# Autodesk Inventor assembly: Assembly
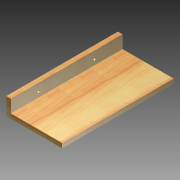
[picture p0: Inventor's stored thumbnail of the model, 180x180]
Saved by Autodesk Inventor 2012 (Build 160160000, 160)
## iProperties
Created: 2013-12-06
Part Number: Assembly
Document SubType Name: Assembly
Designer: PADIAUMESH
Author: PADIAUMESH
## Documents named in this file (3)
- C:\Users\PADIAUMESH\git\AbilityOne\CAD\Assembly.iam
- C:\Users\PADIAUMESH\git\AbilityOne\CAD\base.ipt
- C:\Users\PADIAUMESH\git\AbilityOne\CAD\backboard.ipt
## Components (2 placed, 2 different names)
1. base:1 — Mate:1, Flush:1, Flush:2
2. backboard:1 — Mate:1, Flush:1, Flush:2
## Relationships (3: Flush 2, Mate 1)
- Mate:1: base:1 ↔ backboard:1
- Flush:1: base:1 ↔ backboard:1
- Flush:2: base:1 ↔ backboard:1
